# Autodesk Inventor assembly: POM_T5_03
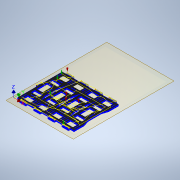
[picture p0: Inventor's stored thumbnail of the model, 180x180]
Saved by Autodesk Inventor 2020 (Build 240168000, 168)
## iProperties
Created: 2021-08-27
Part Number: POM_T5_03
Document SubType Name: Assembly
Designer: Masato
Author: Masato
## Documents named in this file (3)
- C:\Users\naoki\Documents\Inventor\CitBrains\git_clone\SUSTAINA_ver1_0\GFRP\SUSTAINA-OP\Cam\POM_T5_03.iam
- C:\Users\naoki\Documents\Inventor\CitBrains\git_clone\SUSTAINA_ver1_0\GFRP\SUSTAINA-OP\Cam\DisposableBoard.ipt
- C:\Users\naoki\Documents\Inventor\CitBrains\git_clone\SUSTAINA_ver1_0\GFRP\SUSTAINA-OP\UpperBody\Trunk\Trunk_chest_frame.ipt
## Components (5 placed, 2 different names)
1. DisposableBoard:1 — メイト:2, メイト:1, フラッシュ:1, フラッシュ:2, メイト:4, フラッシュ:3, フラッシュ:4
2. Trunk_chest_frame:1 — メイト:4, フラッシュ:3, フラッシュ:4
3. Trunk_chest_frame:3
4. Trunk_chest_frame:4
5. Trunk_chest_frame:5
## Component patterns: (4 elements, first: Trunk_chest_frame:1)
## Relationships (7: Flush 4, Mate 3)
- メイト:2 [Mate]: DisposableBoard:1
- メイト:1 [Mate]: DisposableBoard:1
- フラッシュ:1 [Flush]: DisposableBoard:1
- フラッシュ:2 [Flush]: DisposableBoard:1
- メイト:4 [Mate]: DisposableBoard:1 ↔ Trunk_chest_frame:1
- フラッシュ:3 [Flush] (2 mm): DisposableBoard:1 ↔ Trunk_chest_frame:1
- フラッシュ:4 [Flush] (2 mm): DisposableBoard:1 ↔ Trunk_chest_frame:1
